# Autodesk Inventor assembly: onTelMountingAssy
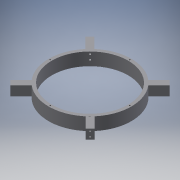
[picture p0: Inventor's stored thumbnail of the model, 180x180]
Saved by Autodesk Inventor 2016 (Build 200138000, 138)
## iProperties
Created: 2015-12-10
Part Number: onTelMountingAssy
Document SubType Name: Assembly
Designer: Dave
Author: Dave
## Documents named in this file (3)
- C:\Users\Dave\Desktop\leuschner-cad\onTelMountingAssy.iam
- C:\Users\Dave\Desktop\leuschner-cad\ontelMounting.ipt
- C:\Users\Dave\Desktop\leuschner-cad\mountingStub.ipt
## Components (5 placed, 2 different names)
1. ontelMounting:1 — Flush:1
2. mountingStub:1 — Flush:1
3. mountingStub:2
4. mountingStub:3
5. mountingStub:4
## Component patterns: (4 elements, first: mountingStub:1)
## Relationships (1: Flush 1)
- Flush:1: ontelMounting:1 ↔ mountingStub:1
